# Autodesk Inventor assembly: NixieClock
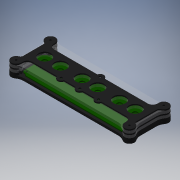
[picture p0: Inventor's stored thumbnail of the model, 180x180]
Saved by Autodesk Inventor 2017 (Build 210142000, 142)
## iProperties
Created: 2017-04-16
Part Number: NixieClock
Document SubType Name: Assembly
Designer: jeffkub
Author: jeffkub
## Documents named in this file (9)
- C:\Projects\nixie-clock\mechanical\NixieClock.iam
- C:\Projects\nixie-clock\mechanical\Base1.ipt
- C:\Projects\nixie-clock\mechanical\Base2.ipt
- C:\Projects\nixie-clock\mechanical\MainPCB.ipt
- C:\Projects\nixie-clock\mechanical\Spacer1.ipt
- C:\Projects\nixie-clock\mechanical\TubePCB.ipt
- C:\Projects\nixie-clock\mechanical\Spacer2.ipt
- C:\Projects\nixie-clock\mechanical\Top.ipt
- C:\Projects\nixie-clock\mechanical\Cover.ipt
## Components (14 placed, 8 different names)
1. Base1:1 — Flush:1, Flush:2, Flush:3, Mate:1
2. Base2:1 — Flush:4, Flush:5, Mate:1, Mate:2, Mate:3, Mate:4, Mate:12, Mate:13
3. MainPCB:1 — Flush:6, Flush:7, Mate:2, Mate:5
4. Spacer1:1 — Mate:3, Mate:4, Angle:1, Mate:6, Mate:8
5. TubePCB:1 — Flush:8, Mate:5, Flush:9
6. Spacer1:2 — Mate:6, Mate:7, Mate:8, Mate:9, Angle:2
7. Spacer2:1 — Mate:7, Mate:9, Angle:3, Mate:10, Mate:11
8. Spacer1:3 — Mate:10, Mate:11, Angle:4
9. Spacer1:4 — Mate:12, Mate:13, Angle:5, Mate:14, Mate:15
10. Spacer1:5 — Mate:14, Mate:15, Angle:6, Mate:16, Mate:17
11. Spacer1:6 — Mate:18, Mate:19, Angle:8, Mate:20
12. Spacer2:2 — Mate:16, Mate:17, Angle:7, Mate:18, Mate:19
13. Top:1 — Mate:20, Flush:10, Flush:11, Mate:21
14. Cover:1 — Mate:21, Flush:12, Flush:13
## Relationships (42: Mate 21, Flush 13, Angle 8)
- Flush:1: Base1:1
- Flush:2: Base1:1
- Flush:3: Base1:1
- Flush:4: Base2:1
- Flush:5: Base2:1
- Mate:1: Base1:1 ↔ Base2:1
- Flush:6: MainPCB:1
- Flush:7: MainPCB:1
- Mate:2: Base2:1 ↔ MainPCB:1
- Mate:3: Base2:1 ↔ Spacer1:1
- Mate:4: Base2:1 ↔ Spacer1:1
- Angle:1 (0 deg): Spacer1:1
- Flush:8: TubePCB:1
- Mate:5 (7.1 mm): MainPCB:1 ↔ TubePCB:1
- Flush:9: TubePCB:1
- Mate:6: Spacer1:1 ↔ Spacer1:2
- Mate:7: Spacer1:2 ↔ Spacer2:1
- Mate:8: Spacer1:1 ↔ Spacer1:2
- Mate:9: Spacer1:2 ↔ Spacer2:1
- Angle:2 (0 deg): Spacer1:2
- Angle:3 (0 deg): Spacer2:1
- Mate:10: Spacer2:1 ↔ Spacer1:3
- Mate:11: Spacer2:1 ↔ Spacer1:3
- Angle:4 (0 deg): Spacer1:3
- Mate:12: Base2:1 ↔ Spacer1:4
- Mate:13: Base2:1 ↔ Spacer1:4
- Angle:5 (0 deg): Spacer1:4
- Mate:14: Spacer1:4 ↔ Spacer1:5
- Mate:15: Spacer1:4 ↔ Spacer1:5
- Angle:6 (0 deg): Spacer1:5
- Mate:16: Spacer1:5 ↔ Spacer2:2
- Mate:17: Spacer1:5 ↔ Spacer2:2
- Angle:7 (0 deg): Spacer2:2
- Mate:18: Spacer1:6 ↔ Spacer2:2
- Mate:19: Spacer1:6 ↔ Spacer2:2
- Angle:8 (0 deg): Spacer1:6
- Mate:20: Spacer1:6 ↔ Top:1
- Flush:10: Top:1
- Flush:11: Top:1
- Mate:21: Top:1 ↔ Cover:1
- Flush:12: Cover:1
- Flush:13: Cover:1
